# Autodesk Inventor assembly: VP-Input-Redline
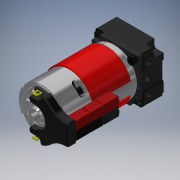
[picture p0: Inventor's stored thumbnail of the model, 180x180]
Saved by Autodesk Inventor 2019 (Build 230136000, 136)
## iProperties
Created: 2018-08-19
Part Number: VP-Input-Redline
Document SubType Name: Assembly
Designer: Rafi
Mass: 464.618 g
Surface Area: 542.341 cm^2
Volume: 76.9621 cm^3
Density: 6.03696 g/cm^3
Author: Rafi
## Documents named in this file (12)
- C:\Users\blairrobotproject\Documents\GrabCAD\Common Parts Library\Gearboxes\Planetary Gearboxes\V2 Stages\V2 Input Stage\VP Redline Input.iam
- C:\Users\blairrobotproject\Documents\GrabCAD\Common Parts Library\Gearboxes\Planetary Gearboxes\V2 Stages\V2 Input Housing.ipt
- C:\Users\blairrobotproject\Documents\GrabCAD\Common Parts Library\Gearboxes\Planetary Gearboxes\Motor Mounting Plates\VP 775 Mounting Plate.ipt
- C:\Users\blairrobotproject\Documents\GrabCAD\Common Parts Library\Gearboxes\Planetary Gearboxes\Screws\M4 x 10mm Screw.ipt
- C:\Users\blairrobotproject\Documents\GrabCAD\Common Parts Library\Motors\Redline.ipt
- C:\Users\blairrobotproject\Documents\GrabCAD\Common Parts Library\Gearboxes\Planetary Gearboxes\Input Coupler\5mm Coupler Sleeve.ipt
- C:\Users\blairrobotproject\Documents\GrabCAD\Common Parts Library\Gearboxes\Planetary Gearboxes\Input Coupler\VP Input Coupler.ipt
- C:\Users\blairrobotproject\Documents\GrabCAD\Common Parts Library\Gearboxes\Planetary Gearboxes\Input Coupler\Coupler Set Screw.ipt
- C:\Users\blairrobotproject\Documents\GrabCAD\Common Parts Library\Gearboxes\Planetary Gearboxes\Screws\8-32 x 0.50in Screw.ipt
- C:\Users\blairrobotproject\Documents\GrabCAD\Common Parts Library\Electronics\Detailed Parts\775 Inline Connector\775_inline_connector_v1.ipt
- C:\Users\blairrobotproject\Documents\GrabCAD\Common Parts Library\Electronics\Detailed Parts\PowerPoles.ipt
- C:\Users\blairrobotproject\Documents\GrabCAD\Common Parts Library\Gearboxes\Planetary Gearboxes\V2 Stages\V2 Input Stage.iam
## Components (12 placed, 10 different names)
1. V2 Input Housing:1 — Mate:1, Mate:2, Flush:1, Mate:13, Flush:5, Mate:14, Mate:15
2. VP 775 Mounting Plate:1 — Mate:1, Mate:2, Flush:1, Insert:1, Insert:2, Insert:7, Insert:8, Mate:17
3. M4 x 10mm Screw:1 — Insert:1
4. M4 x 10mm Screw:2 — Insert:2
5. Redline:1 — Insert:7, Insert:8, Insert:11, Mate:23, Mate:24, Angle:4
6. 5mm Coupler Sleeve:1 — Insert:11, Angle:1
7. VP Input Coupler:1 — Angle:1, Mate:12, Tangent:1, Mate:13, Flush:5
8. Coupler Set Screw:1 — Mate:12, Tangent:1
9. 8-32 x 0.50in Screw:1 — Mate:14, Mate:17, Flush:6
10. 8-32 x 0.50in Screw:2 — Mate:15, Flush:6
11. 775_inline_connector_v1:1 — Mate:23, Mate:24, Angle:4
12. PowerPoles:1
## Relationships (20: Mate 9, Insert 5, Flush 3, Angle 2, Tangent 1)
- Mate:1: V2 Input Housing:1 ↔ VP 775 Mounting Plate:1
- Mate:2: V2 Input Housing:1 ↔ VP 775 Mounting Plate:1
- Flush:1: V2 Input Housing:1 ↔ VP 775 Mounting Plate:1
- Insert:1: VP 775 Mounting Plate:1 ↔ M4 x 10mm Screw:1
- Insert:2: VP 775 Mounting Plate:1 ↔ M4 x 10mm Screw:2
- Insert:7: VP 775 Mounting Plate:1 ↔ Redline:1
- Insert:8: VP 775 Mounting Plate:1 ↔ Redline:1
- Insert:11: Redline:1 ↔ 5mm Coupler Sleeve:1
- Angle:1 (0 deg): 5mm Coupler Sleeve:1 ↔ VP Input Coupler:1
- Mate:12: VP Input Coupler:1 ↔ Coupler Set Screw:1
- Tangent:1: VP Input Coupler:1 ↔ Coupler Set Screw:1
- Mate:13: V2 Input Housing:1 ↔ VP Input Coupler:1
- Flush:5 (2.4 mm): V2 Input Housing:1 ↔ VP Input Coupler:1
- Mate:14: V2 Input Housing:1 ↔ 8-32 x 0.50in Screw:1
- Mate:15: V2 Input Housing:1 ↔ 8-32 x 0.50in Screw:2
- Mate:17: VP 775 Mounting Plate:1 ↔ 8-32 x 0.50in Screw:1
- Flush:6: 8-32 x 0.50in Screw:1 ↔ 8-32 x 0.50in Screw:2
- Mate:23: Redline:1 ↔ 775_inline_connector_v1:1
- Mate:24: Redline:1 ↔ 775_inline_connector_v1:1
- Angle:4 (0 deg): Redline:1 ↔ 775_inline_connector_v1:1
